# Autodesk Inventor assembly: Force_plate
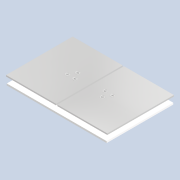
[picture p0: Inventor's stored thumbnail of the model, 180x180]
Saved by Autodesk Inventor 2022 (Build 260153000, 153)
## iProperties
Created: 2023-06-20
Part Number: Force_plate
Document SubType Name: Assembly
Designer: 81805
Author: 81805
## Documents named in this file (5)
- D:\GitHub\inventor\ForcePlate\Force_plate.iam
- D:\GitHub\inventor\ForcePlate\FFS080YS102U6.ipt
- D:\GitHub\inventor\ForcePlate\Board.ipt
- D:\GitHub\inventor\ForcePlate\Bottom_board.ipt
- D:\GitHub\inventor\ForcePlate\M6-14.ipt
## Components (11 placed, 4 different names)
1. FFS080YS102U6:1 — メイト:2, メイト:5, 角度:1, 角度:2, メイト:7
2. FFS080YS102U6:2 — メイト:3, メイト:6, 角度:3, 角度:4, メイト:7
3. Board:1 — メイト:2, フラッシュ:2, フラッシュ:3, 挿入:3, 挿入:4, 挿入:5
4. Board:2 — メイト:3, フラッシュ:1, 挿入:1, 挿入:2, 挿入:6
5. Bottom_board:1 — メイト:5, メイト:6, フラッシュ:1, フラッシュ:2, フラッシュ:3
6. M6-14:1 — 挿入:5
7. M6-14:2 — 挿入:4
8. M6-14:3 — 挿入:6
9. M6-14:4 — 挿入:3
10. M6-14:5 — 挿入:2
11. M6-14:6 — 挿入:1
## Relationships (18: Insert 6, Mate 5, Angle 4, Flush 3)
- メイト:2 [Mate]: FFS080YS102U6:1 ↔ Board:1
- メイト:3 [Mate]: FFS080YS102U6:2 ↔ Board:2
- メイト:5 [Mate]: FFS080YS102U6:1 ↔ Bottom_board:1
- メイト:6 [Mate]: FFS080YS102U6:2 ↔ Bottom_board:1
- フラッシュ:1 [Flush]: Board:2 ↔ Bottom_board:1
- フラッシュ:2 [Flush]: Board:1 ↔ Bottom_board:1
- 角度:1 [Angle] (0 deg): FFS080YS102U6:1
- 角度:2 [Angle] (180 deg): FFS080YS102U6:1
- 角度:3 [Angle] (0 deg): FFS080YS102U6:2
- 角度:4 [Angle] (180 deg): FFS080YS102U6:2
- メイト:7 [Mate] (20 mm): FFS080YS102U6:1 ↔ FFS080YS102U6:2
- フラッシュ:3 [Flush] (-2 mm): Board:1 ↔ Bottom_board:1
- 挿入:1 [Insert]: Board:2 ↔ M6-14:6
- 挿入:2 [Insert]: Board:2 ↔ M6-14:5
- 挿入:3 [Insert]: Board:1 ↔ M6-14:4
- 挿入:4 [Insert]: Board:1 ↔ M6-14:2
- 挿入:5 [Insert]: Board:1 ↔ M6-14:1
- 挿入:6 [Insert]: Board:2 ↔ M6-14:3
